# Autodesk Inventor assembly: wrist_extend
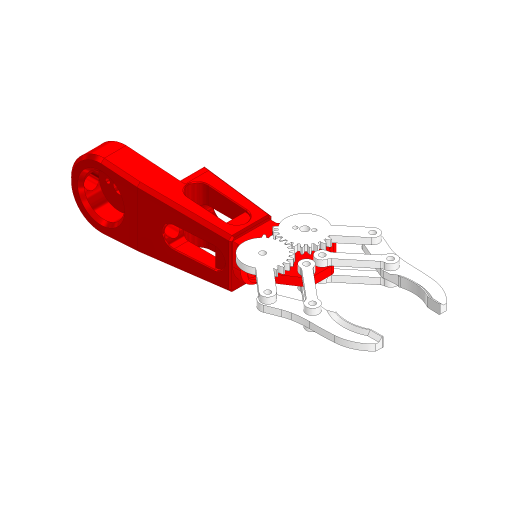
[picture p0: Inventor's stored thumbnail of the model, 512x512]
Saved by Autodesk Inventor 2023 (Build 270158000, 158)
## iProperties
Created: 2023-04-23
Part Number: wrist_extend
Document SubType Name: Assembly
Designer: denyh
Author: denyh
## Documents named in this file (8)
- C:\Users\denyh\Desktop\Rameno\wrist_extend.iam
- C:\Users\denyh\Desktop\Rameno\arm_part3.ipt
- C:\Users\denyh\Desktop\Rameno\grip_base.ipt
- C:\Users\denyh\Desktop\Rameno\lapak2.ipt
- C:\Users\denyh\Desktop\Rameno\lapak.ipt
- C:\Users\denyh\Desktop\Rameno\spojka.ipt
- C:\Users\denyh\Desktop\Rameno\zubate_kolo2.ipt
- C:\Users\denyh\Desktop\Rameno\zubate_kolo1.ipt
## Components (10 placed, 7 different names)
1. arm_part3:1 — Rotational:1
2. grip_base:1 — Rotational:1, Rotational:2, Rotational:3, Rotational:5, Rotational:7, Rotational:8, Rotational:9
3. lapak2:1 — Rotational:10, Mate:3, Mate:4
4. lapak:1 — Rotational:6, Mate:1, Mate:2
5. spojka:1 — Rotational:5, Mate:2
6. spojka:2 — Rotational:7, Mate:1
7. spojka:3 — Rotational:9, Mate:4
8. spojka:4 — Rotational:8, Mate:3
9. zubate_kolo2:1 — Rotational:2, Rotational:6, Rotation:1
10. zubate_kolo1:1 — Rotational:3, Rotational:10, Rotation:1
## Relationships (14: RevoluteJoint 9, Mate 4, RelateRotation 1)
- Rotational:1 [RevoluteJoint]: arm_part3:1 ↔ grip_base:1
- Rotational:2 [RevoluteJoint]: grip_base:1 ↔ zubate_kolo2:1
- Rotational:3 [RevoluteJoint]: grip_base:1 ↔ zubate_kolo1:1
- Rotational:5 [RevoluteJoint]: grip_base:1 ↔ spojka:1
- Rotational:6 [RevoluteJoint]: lapak:1 ↔ zubate_kolo2:1
- Rotational:7 [RevoluteJoint]: grip_base:1 ↔ spojka:2
- Mate:1: lapak:1 ↔ spojka:2
- Mate:2: lapak:1 ↔ spojka:1
- Rotational:8 [RevoluteJoint]: grip_base:1 ↔ spojka:4
- Rotational:9 [RevoluteJoint]: grip_base:1 ↔ spojka:3
- Rotational:10 [RevoluteJoint]: lapak2:1 ↔ zubate_kolo1:1
- Mate:3: lapak2:1 ↔ spojka:4
- Mate:4: lapak2:1 ↔ spojka:3
- Rotation:1 [RelateRotation] (1 ul): zubate_kolo2:1 ↔ zubate_kolo1:1
